# Autodesk Inventor assembly: finalized collector and pan
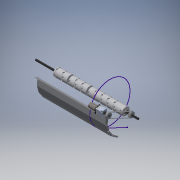
[picture p0: Inventor's stored thumbnail of the model, 180x180]
Saved by Autodesk Inventor 2016 (Build 200138000, 138)
## iProperties
Created: 2017-01-29
Part Number: finalized collector and pan
Document SubType Name: Assembly
Designer: taylorn
Title: C:\Users\nick pc\Desktop\git hub robotics\finalized collector and pan.stp
Author: nick pc
Sending System: Autodesk Inventor 2015
Preprocessor: ST-DEVELOPER v15.6
## Documents named in this file (7)
- D:\1073CAD\Robot2017\finalized collector and pan.iam
- D:\1073CAD\Robot2017\plate.ipt
- D:\1073CAD\Robot2017\BRUCES ROLLER.ipt
- D:\1073CAD\Robot2017\.5 HEX BEARING.ipt
- D:\1073CAD\Robot2017\thunder hex.ipt
- D:\1073CAD\Robot2017\belts and pullys.iam
- D:\1073CAD\Robot2017\v2-VersaPlanetary-1stage-with-AM9015-20131031.iam
## Components (7 placed, 6 different names)
1. plate:1
2. BRUCES ROLLER:1
3. .5 HEX BEARING:1
4. .5 HEX BEARING:2
5. thunder hex:1 — Mate:1
6. belts and pullys:1 [sub-assembly] — Mate:1, Mate:2, Mate:3
7. v2-VersaPlanetary-1stage-with-AM9015-20131031:1 [sub-assembly] — Mate:2, Mate:3
## Relationships (3: Mate 3)
- Mate:1: thunder hex:1 ↔ belts and pullys:1
- Mate:2: belts and pullys:1 ↔ v2-VersaPlanetary-1stage-with-AM9015-20131031:1
- Mate:3: belts and pullys:1 ↔ v2-VersaPlanetary-1stage-with-AM9015-20131031:1
